# Autodesk Inventor assembly: 000-dribl-v2
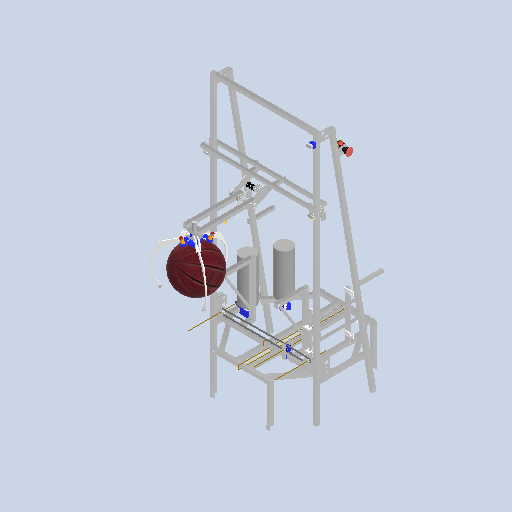
[picture p0: Inventor's stored thumbnail of the model, 512x512]
Saved by Autodesk Inventor 2025.2 (Build 292293000, 293)
## iProperties
Created: 2025-04-03
Part Number: 000-dribl-v2
Document SubType Name: Assembly
Designer: haruy
Author: haruy
## Documents named in this file (45)
- C:\Users\haruy\Documents\ロボコン\NHK2025\cad\nagahisa\dribl\000-dribl-v2.iam
- C:\Users\haruy\Documents\ロボコン\NHK2025\cad\nagahisa\dribl\dribl-v3-Sketch-Base.ipt
- C:\Users\haruy\Documents\ロボコン\NHK2025\cad\nagahisa\dribl\dribl-v1-Plate-5.ipt
- C:\Users\haruy\Documents\ロボコン\NHK2025\cad\nagahisa\dribl\dribl-v1-Plate-3.ipt
- C:\Users\haruy\Documents\ロボコン\NHK2025\cad\nagahisa\dribl\dribl-v1-Plate-4.ipt
- C:\Users\haruy\Documents\ロボコン\NHK2025\cad\nagahisa\dribl\dribl-v3-Plate-1.ipt
- C:\Users\haruy\Documents\ロボコン\NHK2025\cad\nagahisa\dribl\dribl-v3-Plate-2.ipt
- C:\Users\haruy\Documents\ロボコン\NHK2025\cad\nagahisa\dribl\dribl-v3-ASP-arm.ipt
- C:\Users\haruy\Documents\ロボコン\NHK2025\cad\nagahisa\dribl\dribl-v3-Plate-3.ipt
- C:\Users\haruy\Documents\ロボコン\NHK2025\cad\nagahisa\dribl\dribl-v1-Shaft-spesa-57.ipt
- C:\Users\haruy\Documents\ロボコン\NHK2025\cad\nagahisa\dribl\dribl-v3-Plate-4.ipt
- C:\Users\haruy\Documents\ロボコン\NHK2025\cad\nagahisa\dribl\dribl-v1-Plate-8.ipt
- C:\Users\haruy\Documents\ロボコン\NHK2025\cad\000_parts\モーター\robomaster\M2006 P36\RoboMaster M2006 P36\RoboMaster M2006 P36.ipt
- C:\Users\haruy\Documents\ロボコン\NHK2025\cad\nagahisa\dribl\dribl-v3-Plate-6.ipt
- C:\Users\haruy\Documents\ロボコン\NHK2025\cad\nagahisa\dribl\dribl-v3-Plate-7.ipt
- C:\Users\haruy\Documents\ロボコン\NHK2025\cad\nagahisa\dribl\dribl-v3-Plate-8.ipt
- C:\Users\haruy\Documents\ロボコン\NHK2025\cad\nagahisa\dribl\dribl-v3-Plate-9.ipt
- C:\Users\haruy\Documents\ロボコン\NHK2025\cad\nagahisa\dribl\dribl-v3-Plate-10.ipt
- C:\Users\haruy\Documents\ロボコン\NHK2025\cad\nagahisa\dribl\dribl-v3-Plate-11.ipt
- C:\Users\haruy\Documents\ロボコン\NHK2025\cad\nagahisa\dribl\dribl-v3-Plate-12.ipt
- C:\Users\haruy\Documents\ロボコン\NHK2025\cad\nagahisa\dribl\dribl-v3-ASP-1.ipt
- C:\Users\haruy\Documents\ロボコン\NHK2025\cad\nagahisa\dribl\dribl-v1-Plate-14.ipt
- C:\Users\haruy\Documents\ロボコン\NHK2025\cad\nagahisa\dribl\dribl-v1-3DP-P-F.ipt
- C:\Users\haruy\Documents\ロボコン\NHK2025\cad\nagahisa\dribl\roller-Base-v1-petbottle.ipt
- C:\Users\haruy\Documents\ロボコン\NHK2025\cad\nagahisa\dribl\dribl-v3-Plate-13.ipt
- C:\Users\haruy\Documents\ロボコン\NHK2025\cad\nagahisa\dribl\dribl-v3-Plate-14.ipt
- C:\Users\haruy\Documents\ロボコン\NHK2025\cad\nagahisa\base_weel\base_weel-v2-Plate-8.ipt
- C:\Users\haruy\Documents\ロボコン\NHK2025\cad\nagahisa\dribl\dribl-v3-ASP-2.ipt
- C:\Users\haruy\Documents\ロボコン\NHK2025\cad\nagahisa\base_weel\base_weel-v2-POM-pc-F-1.ipt
- C:\Users\haruy\Documents\ロボコン\NHK2025\cad\nagahisa\base_weel\base_weel-v2-POM-pc-F-2.ipt
- C:\Users\haruy\Documents\ロボコン\NHK2025\cad\nagahisa\dribl\dribl-v3-Plate-15.ipt
- C:\Users\haruy\Documents\ロボコン\NHK2025\cad\nagahisa\dribl\dribl-v1-Plate-13.ipt
- C:\Users\haruy\Documents\ロボコン\NHK2025\cad\000_parts\回路関連\EMO\emo_sa.ipt
- C:\Users\haruy\Documents\ロボコン\NHK2025\cad\nagahisa\dribl\dribl-v3-3DP-1.ipt
- C:\Users\haruy\Documents\ロボコン\NHK2025\cad\nagahisa\dribl\dribl-v3-Plate-16.ipt
- C:\Users\haruy\Documents\ロボコン\NHK2025\cad\nagahisa\dribl\000-dribl-v2\デザイン アクセラレータ\歯付きベルト伝達1.iam
- C:\Users\haruy\Documents\ロボコン\NHK2025\cad\000_parts\ベアリング\10\bear_10_15_sn.ipt
- C:\Users\haruy\Documents\ロボコン\NHK2025\cad\nagahisa\belt_liner\SCBRJ10-13.iam
- C:\Users\haruy\Documents\ロボコン\NHK2025\cad\nagahisa\dribl\dribl-v1-Plate-12.ipt
- C:\Users\haruy\Documents\ロボコン\NHK2025\cad\nagahisa\dribl\dribl-v1-3DP-l-F-1.ipt
- C:\Users\haruy\Documents\ロボコン\NHK2025\cad\000_parts\センサー\VX-012-1A3\VX-012-1A3\VX-012-1A3.iam
- C:\Users\haruy\Documents\ロボコン\NHK2025\cad\nagahisa\dribl\R2-Rzvector\TH22_bearing_12_18_19.5_sn.ipt
- C:\Users\haruy\Documents\ロボコン\NHK2025\cad\nagahisa\dribl\SCSNAJ12-16b.ipt
- C:\Users\haruy\Documents\ロボコン\NHK2025\cad\nagahisa\dribl\dribl-v1-Shaft-2.ipt
- C:\Users\haruy\Documents\ロボコン\NHK2025\cad\nagahisa\hand\grab\000-hand-grab-v4.iam
## Components (87 placed, 44 different names)
1. dribl-v3-Sketch-Base:1 — 挿入:10, 挿入:11, 挿入:12, 挿入:13, 挿入:14, 挿入:15, 挿入:16, 挿入:17, 挿入:18, 挿入:19, 挿入:20, 挿入:21, 挿入:22, 挿入:23, 挿入:24, 挿入:25, 挿入:26, 挿入:27, 挿入:28, 挿入:29, 挿入:30, 挿入:31, 挿入:32, 挿入:33, 正接:1, 正接:2, 正接:3, 正接:4, 挿入:44, 挿入:45, 挿入:46, 挿入:47, 挿入:48, 挿入:49, 挿入:50, 挿入:51, 挿入:52, 挿入:53, 挿入:56, 挿入:57, 挿入:58, 挿入:59, 挿入:60, 挿入:61, 挿入:62, 挿入:63, 挿入:64, 挿入:65, 挿入:70, 挿入:71, 挿入:72, 挿入:73, 挿入:74, 挿入:75, 挿入:76, 挿入:77, 挿入:78, 挿入:79, 挿入:80, 挿入:81, 挿入:82, 挿入:83, 挿入:84, 挿入:85, 挿入:86, 挿入:87, 挿入:88, 挿入:89, 挿入:90, 挿入:91, 挿入:92, 挿入:93, 挿入:94, 挿入:95, 挿入:96, 挿入:97, メイト:3, メイト:4, メイト:5, メイト:6, 挿入:102, 挿入:103, 挿入:104, 挿入:105, 挿入:106, 挿入:107, 挿入:108, 挿入:109, 挿入:128, 挿入:129, 挿入:130, 挿入:131, 挿入:132, 挿入:133, 挿入:134, 挿入:135, 挿入:137, 挿入:138, 挿入:139, 挿入:140, フラッシュ:1, 挿入:149, 挿入:150, 挿入:151, 挿入:152
2. dribl-v1-Plate-5:1 — 挿入:12, 挿入:13
3. dribl-v1-Plate-5:2 — 挿入:10, 挿入:11
4. dribl-v1-Plate-3:1 — 挿入:14, 挿入:15
5. dribl-v1-Plate-4:1 — 挿入:16, 挿入:17
6. dribl-v3-Plate-1:1 — 挿入:18, 挿入:19
7. dribl-v3-Plate-1:2 — 挿入:20, 挿入:21
8. dribl-v3-Plate-1:3 — 挿入:22, 挿入:23
9. dribl-v3-Plate-1:4 — 挿入:24, 挿入:25
10. dribl-v3-Plate-2:1 — 挿入:26, 挿入:27
11. dribl-v3-Plate-2:2 — 挿入:28, 挿入:29
12. dribl-v3-Plate-2:3 — 挿入:32, 挿入:33
13. dribl-v3-Plate-2:4 — 挿入:30, 挿入:31
14. dribl-v3-ASP-arm:1 — 正接:1, 正接:2, 正接:3, 正接:4, 挿入:34, 挿入:35, 挿入:37, 挿入:38, メイト:7, 角度:1
15. dribl-v3-Plate-3:1 — 挿入:34, 挿入:35, 挿入:36, 挿入:39, 挿入:40, 挿入:158
16. dribl-v1-Shaft-spesa-57:1 — 挿入:36, 挿入:41
17. dribl-v3-Plate-4:1 — 挿入:37, 挿入:38, 挿入:157
18. dribl-v1-Shaft-spesa-57:2 — 挿入:40
19. dribl-v1-Shaft-spesa-57:3 — 挿入:39, 挿入:42
20. dribl-v1-Plate-8:1 — 挿入:41, 挿入:42, 挿入:43
21. RoboMaster M2006 P36:1 — 挿入:43
22. dribl-v3-Plate-6:1 — 挿入:44, 挿入:45
23. dribl-v3-Plate-6:2 — 挿入:50, 挿入:51
24. dribl-v3-Plate-6:3 — 挿入:48, 挿入:49
25. dribl-v3-Plate-6:4 — 挿入:46, 挿入:47
26. dribl-v3-Plate-7:1 — 挿入:52, 挿入:53
27. dribl-v3-Plate-7:4 — 挿入:56, 挿入:57
28. dribl-v3-Plate-8:1 — 挿入:58, 挿入:59
29. dribl-v3-Plate-8:2 — 挿入:60, 挿入:61
30. dribl-v3-Plate-9:1 — 挿入:62, 挿入:63
31. dribl-v3-Plate-9:3 — 挿入:64, 挿入:65
32. dribl-v3-Plate-10:1 — 挿入:72, 挿入:73
33. dribl-v3-Plate-10:2 — 挿入:74, 挿入:75
34. dribl-v3-Plate-10:3 — 挿入:70, 挿入:71
35. dribl-v3-Plate-10:4 — 挿入:76, 挿入:77
36. dribl-v3-Plate-11:1 — 挿入:78, 挿入:79
37. dribl-v3-Plate-11:2 — 挿入:82, 挿入:83
38. dribl-v3-Plate-11:3 — 挿入:80, 挿入:81
39. dribl-v3-Plate-11:4 — 挿入:84, 挿入:85
40. dribl-v3-Plate-11:5 — 挿入:88, 挿入:89
41. dribl-v3-Plate-11:6 — 挿入:86, 挿入:87
42. dribl-v3-Plate-12:1 — 挿入:90, 挿入:91
43. dribl-v3-Plate-12:2 — 挿入:92, 挿入:93
44. dribl-v3-ASP-1:1 — 挿入:98, 挿入:99
45. dribl-v1-Plate-14:1 — 挿入:96, 挿入:97
46. dribl-v1-Plate-14:2 — 挿入:94, 挿入:95, 挿入:98, 挿入:99
47. dribl-v1-3DP-P-F:1 — 挿入:100, メイト:5, メイト:6
48. roller-Base-v1-petbottle:1 — 挿入:100
49. dribl-v1-3DP-P-F:2 — メイト:3, メイト:4, 挿入:101
50. roller-Base-v1-petbottle:2 — 挿入:101
51. dribl-v3-Plate-13:1 — 挿入:102, 挿入:103
52. dribl-v3-Plate-14:1 — 挿入:104, 挿入:105
53. base_weel-v2-Plate-8:1 — 挿入:106, 挿入:107, 挿入:110, 挿入:111
54. base_weel-v2-Plate-8:2 — 挿入:108, 挿入:109
55. dribl-v3-ASP-2:1 — 挿入:110, 挿入:111, 挿入:112, 挿入:113, 挿入:114, 挿入:115, 挿入:116, 挿入:117, 挿入:118, 挿入:119, 挿入:120, 挿入:121, 挿入:122, 挿入:123, 挿入:124, 挿入:125, 挿入:126, 挿入:127
56. base_weel-v2-POM-pc-F-1:1 — 挿入:112, 挿入:113
57. base_weel-v2-POM-pc-F-1:2 — 挿入:114, 挿入:115
58. base_weel-v2-POM-pc-F-2:1 — 挿入:118, 挿入:119
59. base_weel-v2-POM-pc-F-2:2 — 挿入:116, 挿入:117
60. base_weel-v2-POM-pc-F-2:3 — 挿入:122, 挿入:123
61. base_weel-v2-POM-pc-F-2:4 — 挿入:120, 挿入:121
62. base_weel-v2-POM-pc-F-1:3 — 挿入:126, 挿入:127
63. base_weel-v2-POM-pc-F-1:4 — 挿入:124, 挿入:125
64. dribl-v3-Plate-15:1 — 挿入:128, 挿入:129
65. dribl-v3-Plate-15:2 — 挿入:130, 挿入:131
66. dribl-v3-Plate-11:7 — 挿入:132, 挿入:133
67. dribl-v1-Plate-13:1 — 挿入:134, 挿入:135, 挿入:136
68. emo_sa:1 — 挿入:136
69. dribl-v3-3DP-1:1 — 挿入:139, 挿入:140, 挿入:143, 挿入:144
70. dribl-v3-3DP-1:2 — 挿入:137, 挿入:138, 挿入:141, 挿入:142
71. dribl-v3-Plate-16:1 — 挿入:143, 挿入:144
72. dribl-v3-Plate-16:2 — 挿入:141, 挿入:142
73. 歯付きベルト伝達:1 [sub-assembly] — 挿入:145, 挿入:146
74. bear_10_15_sn:1 — 挿入:145, 挿入:147
75. bear_10_15_sn:2 — 挿入:146, 挿入:148
76. SCBRJ10-13:1 [sub-assembly] — 挿入:147
77. SCBRJ10-13:2 [sub-assembly] — 挿入:148
78. dribl-v1-Plate-12:1 — 挿入:149, 挿入:150, 挿入:155, 挿入:156
79. dribl-v1-3DP-l-F-1:1 — 挿入:151, 挿入:152, 挿入:153, 挿入:154
80. VX-012-1A3:1 [sub-assembly] — 挿入:153, 挿入:154
81. VX-012-1A3:2 [sub-assembly] — 挿入:155, 挿入:156, メイト:7
82. TH22_bearing_12_18_19.5_sn:1 — 挿入:157, 挿入:160
83. TH22_bearing_12_18_19.5_sn:2 — 挿入:158, 挿入:159, 挿入:162
84. SCSNAJ12-16b:1 — 挿入:159, 挿入:161
85. SCSNAJ12-16b:2 — 挿入:160
86. dribl-v1-Shaft-2:1 — 挿入:161
87. 000-hand-grab-v4:1 [sub-assembly] — 挿入:162, 角度:1
## Relationships (158: Insert 147, Mate 5, Tangent 4, Flush 1, Angle 1)
- 挿入:10 [Insert]: dribl-v3-Sketch-Base:1 ↔ dribl-v1-Plate-5:2
- 挿入:11 [Insert]: dribl-v3-Sketch-Base:1 ↔ dribl-v1-Plate-5:2
- 挿入:12 [Insert]: dribl-v3-Sketch-Base:1 ↔ dribl-v1-Plate-5:1
- 挿入:13 [Insert]: dribl-v3-Sketch-Base:1 ↔ dribl-v1-Plate-5:1
- 挿入:14 [Insert]: dribl-v3-Sketch-Base:1 ↔ dribl-v1-Plate-3:1
- 挿入:15 [Insert]: dribl-v3-Sketch-Base:1 ↔ dribl-v1-Plate-3:1
- 挿入:16 [Insert]: dribl-v3-Sketch-Base:1 ↔ dribl-v1-Plate-4:1
- 挿入:17 [Insert]: dribl-v3-Sketch-Base:1 ↔ dribl-v1-Plate-4:1
- 挿入:18 [Insert]: dribl-v3-Sketch-Base:1 ↔ dribl-v3-Plate-1:1
- 挿入:19 [Insert]: dribl-v3-Sketch-Base:1 ↔ dribl-v3-Plate-1:1
- 挿入:20 [Insert]: dribl-v3-Sketch-Base:1 ↔ dribl-v3-Plate-1:2
- 挿入:21 [Insert]: dribl-v3-Sketch-Base:1 ↔ dribl-v3-Plate-1:2
- 挿入:22 [Insert]: dribl-v3-Sketch-Base:1 ↔ dribl-v3-Plate-1:3
- 挿入:23 [Insert]: dribl-v3-Sketch-Base:1 ↔ dribl-v3-Plate-1:3
- 挿入:24 [Insert]: dribl-v3-Sketch-Base:1 ↔ dribl-v3-Plate-1:4
- 挿入:25 [Insert]: dribl-v3-Sketch-Base:1 ↔ dribl-v3-Plate-1:4
- 挿入:26 [Insert]: dribl-v3-Sketch-Base:1 ↔ dribl-v3-Plate-2:1
- 挿入:27 [Insert]: dribl-v3-Sketch-Base:1 ↔ dribl-v3-Plate-2:1
- 挿入:28 [Insert]: dribl-v3-Sketch-Base:1 ↔ dribl-v3-Plate-2:2
- 挿入:29 [Insert]: dribl-v3-Sketch-Base:1 ↔ dribl-v3-Plate-2:2
- 挿入:30 [Insert]: dribl-v3-Sketch-Base:1 ↔ dribl-v3-Plate-2:4
- 挿入:31 [Insert]: dribl-v3-Sketch-Base:1 ↔ dribl-v3-Plate-2:4
- 挿入:32 [Insert]: dribl-v3-Sketch-Base:1 ↔ dribl-v3-Plate-2:3
- 挿入:33 [Insert]: dribl-v3-Sketch-Base:1 ↔ dribl-v3-Plate-2:3
- 正接:1 [Tangent]: dribl-v3-Sketch-Base:1 ↔ dribl-v3-ASP-arm:1
- 正接:2 [Tangent]: dribl-v3-Sketch-Base:1 ↔ dribl-v3-ASP-arm:1
- 正接:3 [Tangent]: dribl-v3-Sketch-Base:1 ↔ dribl-v3-ASP-arm:1
- 正接:4 [Tangent]: dribl-v3-Sketch-Base:1 ↔ dribl-v3-ASP-arm:1
- 挿入:34 [Insert]: dribl-v3-ASP-arm:1 ↔ dribl-v3-Plate-3:1
- 挿入:35 [Insert]: dribl-v3-ASP-arm:1 ↔ dribl-v3-Plate-3:1
- 挿入:36 [Insert]: dribl-v3-Plate-3:1 ↔ dribl-v1-Shaft-spesa-57:1
- 挿入:37 [Insert]: dribl-v3-ASP-arm:1 ↔ dribl-v3-Plate-4:1
- 挿入:38 [Insert]: dribl-v3-ASP-arm:1 ↔ dribl-v3-Plate-4:1
- 挿入:39 [Insert]: dribl-v3-Plate-3:1 ↔ dribl-v1-Shaft-spesa-57:3
- 挿入:40 [Insert]: dribl-v3-Plate-3:1 ↔ dribl-v1-Shaft-spesa-57:2
- 挿入:41 [Insert]: dribl-v1-Shaft-spesa-57:1 ↔ dribl-v1-Plate-8:1
- 挿入:42 [Insert]: dribl-v1-Shaft-spesa-57:3 ↔ dribl-v1-Plate-8:1
- 挿入:43 [Insert]: dribl-v1-Plate-8:1 ↔ RoboMaster M2006 P36:1
- 挿入:44 [Insert]: dribl-v3-Sketch-Base:1 ↔ dribl-v3-Plate-6:1
- 挿入:45 [Insert]: dribl-v3-Sketch-Base:1 ↔ dribl-v3-Plate-6:1
- 挿入:46 [Insert]: dribl-v3-Sketch-Base:1 ↔ dribl-v3-Plate-6:4
- 挿入:47 [Insert]: dribl-v3-Sketch-Base:1 ↔ dribl-v3-Plate-6:4
- 挿入:48 [Insert]: dribl-v3-Sketch-Base:1 ↔ dribl-v3-Plate-6:3
- 挿入:49 [Insert]: dribl-v3-Sketch-Base:1 ↔ dribl-v3-Plate-6:3
- 挿入:50 [Insert]: dribl-v3-Sketch-Base:1 ↔ dribl-v3-Plate-6:2
- 挿入:51 [Insert]: dribl-v3-Sketch-Base:1 ↔ dribl-v3-Plate-6:2
- 挿入:52 [Insert]: dribl-v3-Sketch-Base:1 ↔ dribl-v3-Plate-7:1
- 挿入:53 [Insert]: dribl-v3-Sketch-Base:1 ↔ dribl-v3-Plate-7:1
- 挿入:56 [Insert]: dribl-v3-Sketch-Base:1 ↔ dribl-v3-Plate-7:4
- 挿入:57 [Insert]: dribl-v3-Sketch-Base:1 ↔ dribl-v3-Plate-7:4
- 挿入:58 [Insert]: dribl-v3-Sketch-Base:1 ↔ dribl-v3-Plate-8:1
- 挿入:59 [Insert]: dribl-v3-Sketch-Base:1 ↔ dribl-v3-Plate-8:1
- 挿入:60 [Insert]: dribl-v3-Sketch-Base:1 ↔ dribl-v3-Plate-8:2
- 挿入:61 [Insert]: dribl-v3-Sketch-Base:1 ↔ dribl-v3-Plate-8:2
- 挿入:62 [Insert]: dribl-v3-Sketch-Base:1 ↔ dribl-v3-Plate-9:1
- 挿入:63 [Insert]: dribl-v3-Sketch-Base:1 ↔ dribl-v3-Plate-9:1
- 挿入:64 [Insert]: dribl-v3-Sketch-Base:1 ↔ dribl-v3-Plate-9:3
- 挿入:65 [Insert]: dribl-v3-Sketch-Base:1 ↔ dribl-v3-Plate-9:3
- 挿入:70 [Insert]: dribl-v3-Sketch-Base:1 ↔ dribl-v3-Plate-10:3
- 挿入:71 [Insert]: dribl-v3-Sketch-Base:1 ↔ dribl-v3-Plate-10:3
- 挿入:72 [Insert]: dribl-v3-Sketch-Base:1 ↔ dribl-v3-Plate-10:1
- 挿入:73 [Insert]: dribl-v3-Sketch-Base:1 ↔ dribl-v3-Plate-10:1
- 挿入:74 [Insert]: dribl-v3-Sketch-Base:1 ↔ dribl-v3-Plate-10:2
- 挿入:75 [Insert]: dribl-v3-Sketch-Base:1 ↔ dribl-v3-Plate-10:2
- 挿入:76 [Insert]: dribl-v3-Sketch-Base:1 ↔ dribl-v3-Plate-10:4
- 挿入:77 [Insert]: dribl-v3-Sketch-Base:1 ↔ dribl-v3-Plate-10:4
- 挿入:78 [Insert]: dribl-v3-Sketch-Base:1 ↔ dribl-v3-Plate-11:1
- 挿入:79 [Insert]: dribl-v3-Sketch-Base:1 ↔ dribl-v3-Plate-11:1
- 挿入:80 [Insert]: dribl-v3-Sketch-Base:1 ↔ dribl-v3-Plate-11:3
- 挿入:81 [Insert]: dribl-v3-Sketch-Base:1 ↔ dribl-v3-Plate-11:3
- 挿入:82 [Insert]: dribl-v3-Sketch-Base:1 ↔ dribl-v3-Plate-11:2
- 挿入:83 [Insert]: dribl-v3-Sketch-Base:1 ↔ dribl-v3-Plate-11:2
- 挿入:84 [Insert]: dribl-v3-Sketch-Base:1 ↔ dribl-v3-Plate-11:4
- 挿入:85 [Insert]: dribl-v3-Sketch-Base:1 ↔ dribl-v3-Plate-11:4
- 挿入:86 [Insert]: dribl-v3-Sketch-Base:1 ↔ dribl-v3-Plate-11:6
- 挿入:87 [Insert]: dribl-v3-Sketch-Base:1 ↔ dribl-v3-Plate-11:6
- 挿入:88 [Insert]: dribl-v3-Sketch-Base:1 ↔ dribl-v3-Plate-11:5
- 挿入:89 [Insert]: dribl-v3-Sketch-Base:1 ↔ dribl-v3-Plate-11:5
- 挿入:90 [Insert]: dribl-v3-Sketch-Base:1 ↔ dribl-v3-Plate-12:1
- 挿入:91 [Insert]: dribl-v3-Sketch-Base:1 ↔ dribl-v3-Plate-12:1
- 挿入:92 [Insert]: dribl-v3-Sketch-Base:1 ↔ dribl-v3-Plate-12:2
- 挿入:93 [Insert]: dribl-v3-Sketch-Base:1 ↔ dribl-v3-Plate-12:2
- 挿入:94 [Insert]: dribl-v3-Sketch-Base:1 ↔ dribl-v1-Plate-14:2
- 挿入:95 [Insert]: dribl-v3-Sketch-Base:1 ↔ dribl-v1-Plate-14:2
- 挿入:96 [Insert]: dribl-v3-Sketch-Base:1 ↔ dribl-v1-Plate-14:1
- 挿入:97 [Insert]: dribl-v3-Sketch-Base:1 ↔ dribl-v1-Plate-14:1
- 挿入:98 [Insert]: dribl-v3-ASP-1:1 ↔ dribl-v1-Plate-14:2
- 挿入:99 [Insert]: dribl-v3-ASP-1:1 ↔ dribl-v1-Plate-14:2
- 挿入:100 [Insert]: dribl-v1-3DP-P-F:1 ↔ roller-Base-v1-petbottle:1
- メイト:3 [Mate]: dribl-v3-Sketch-Base:1 ↔ dribl-v1-3DP-P-F:2
- メイト:4 [Mate]: dribl-v3-Sketch-Base:1 ↔ dribl-v1-3DP-P-F:2
- 挿入:101 [Insert]: dribl-v1-3DP-P-F:2 ↔ roller-Base-v1-petbottle:2
- メイト:5 [Mate]: dribl-v3-Sketch-Base:1 ↔ dribl-v1-3DP-P-F:1
- メイト:6 [Mate]: dribl-v3-Sketch-Base:1 ↔ dribl-v1-3DP-P-F:1
- 挿入:102 [Insert]: dribl-v3-Sketch-Base:1 ↔ dribl-v3-Plate-13:1
- 挿入:103 [Insert]: dribl-v3-Sketch-Base:1 ↔ dribl-v3-Plate-13:1
- 挿入:104 [Insert]: dribl-v3-Sketch-Base:1 ↔ dribl-v3-Plate-14:1
- 挿入:105 [Insert]: dribl-v3-Sketch-Base:1 ↔ dribl-v3-Plate-14:1
- 挿入:106 [Insert]: dribl-v3-Sketch-Base:1 ↔ base_weel-v2-Plate-8:1
- 挿入:107 [Insert]: dribl-v3-Sketch-Base:1 ↔ base_weel-v2-Plate-8:1
- 挿入:108 [Insert]: dribl-v3-Sketch-Base:1 ↔ base_weel-v2-Plate-8:2
- 挿入:109 [Insert]: dribl-v3-Sketch-Base:1 ↔ base_weel-v2-Plate-8:2
- 挿入:110 [Insert]: base_weel-v2-Plate-8:1 ↔ dribl-v3-ASP-2:1
- 挿入:111 [Insert]: base_weel-v2-Plate-8:1 ↔ dribl-v3-ASP-2:1
- 挿入:112 [Insert]: dribl-v3-ASP-2:1 ↔ base_weel-v2-POM-pc-F-1:1
- 挿入:113 [Insert]: dribl-v3-ASP-2:1 ↔ base_weel-v2-POM-pc-F-1:1
- 挿入:114 [Insert]: dribl-v3-ASP-2:1 ↔ base_weel-v2-POM-pc-F-1:2
- 挿入:115 [Insert]: dribl-v3-ASP-2:1 ↔ base_weel-v2-POM-pc-F-1:2
- 挿入:116 [Insert]: dribl-v3-ASP-2:1 ↔ base_weel-v2-POM-pc-F-2:2
- 挿入:117 [Insert]: dribl-v3-ASP-2:1 ↔ base_weel-v2-POM-pc-F-2:2
- 挿入:118 [Insert]: dribl-v3-ASP-2:1 ↔ base_weel-v2-POM-pc-F-2:1
- 挿入:119 [Insert]: dribl-v3-ASP-2:1 ↔ base_weel-v2-POM-pc-F-2:1
- 挿入:120 [Insert]: dribl-v3-ASP-2:1 ↔ base_weel-v2-POM-pc-F-2:4
- 挿入:121 [Insert]: dribl-v3-ASP-2:1 ↔ base_weel-v2-POM-pc-F-2:4
- 挿入:122 [Insert]: dribl-v3-ASP-2:1 ↔ base_weel-v2-POM-pc-F-2:3
- 挿入:123 [Insert]: dribl-v3-ASP-2:1 ↔ base_weel-v2-POM-pc-F-2:3
- 挿入:124 [Insert]: dribl-v3-ASP-2:1 ↔ base_weel-v2-POM-pc-F-1:4
- 挿入:125 [Insert]: dribl-v3-ASP-2:1 ↔ base_weel-v2-POM-pc-F-1:4
- 挿入:126 [Insert]: dribl-v3-ASP-2:1 ↔ base_weel-v2-POM-pc-F-1:3
- 挿入:127 [Insert]: dribl-v3-ASP-2:1 ↔ base_weel-v2-POM-pc-F-1:3
- 挿入:128 [Insert]: dribl-v3-Sketch-Base:1 ↔ dribl-v3-Plate-15:1
- 挿入:129 [Insert]: dribl-v3-Sketch-Base:1 ↔ dribl-v3-Plate-15:1
- 挿入:130 [Insert]: dribl-v3-Sketch-Base:1 ↔ dribl-v3-Plate-15:2
- 挿入:131 [Insert]: dribl-v3-Sketch-Base:1 ↔ dribl-v3-Plate-15:2
- 挿入:132 [Insert]: dribl-v3-Sketch-Base:1 ↔ dribl-v3-Plate-11:7
- 挿入:133 [Insert]: dribl-v3-Sketch-Base:1 ↔ dribl-v3-Plate-11:7
- 挿入:134 [Insert]: dribl-v3-Sketch-Base:1 ↔ dribl-v1-Plate-13:1
- 挿入:135 [Insert]: dribl-v3-Sketch-Base:1 ↔ dribl-v1-Plate-13:1
- 挿入:136 [Insert]: dribl-v1-Plate-13:1 ↔ emo_sa:1
- 挿入:137 [Insert]: dribl-v3-Sketch-Base:1 ↔ dribl-v3-3DP-1:2
- 挿入:138 [Insert]: dribl-v3-Sketch-Base:1 ↔ dribl-v3-3DP-1:2
- 挿入:139 [Insert]: dribl-v3-Sketch-Base:1 ↔ dribl-v3-3DP-1:1
- 挿入:140 [Insert]: dribl-v3-Sketch-Base:1 ↔ dribl-v3-3DP-1:1
- 挿入:141 [Insert]: dribl-v3-3DP-1:2 ↔ dribl-v3-Plate-16:2
- 挿入:142 [Insert]: dribl-v3-3DP-1:2 ↔ dribl-v3-Plate-16:2
- 挿入:143 [Insert]: dribl-v3-3DP-1:1 ↔ dribl-v3-Plate-16:1
- 挿入:144 [Insert]: dribl-v3-3DP-1:1 ↔ dribl-v3-Plate-16:1
- フラッシュ:1 [Flush] (-10 mm): dribl-v3-Sketch-Base:1
- 挿入:145 [Insert]: 歯付きベルト伝達:1 ↔ bear_10_15_sn:1
- 挿入:146 [Insert]: 歯付きベルト伝達:1 ↔ bear_10_15_sn:2
- 挿入:147 [Insert]: bear_10_15_sn:1 ↔ SCBRJ10-13:1
- 挿入:148 [Insert]: bear_10_15_sn:2 ↔ SCBRJ10-13:2
- 挿入:149 [Insert]: dribl-v3-Sketch-Base:1 ↔ dribl-v1-Plate-12:1
- 挿入:150 [Insert]: dribl-v3-Sketch-Base:1 ↔ dribl-v1-Plate-12:1
- 挿入:151 [Insert]: dribl-v3-Sketch-Base:1 ↔ dribl-v1-3DP-l-F-1:1
- 挿入:152 [Insert]: dribl-v3-Sketch-Base:1 ↔ dribl-v1-3DP-l-F-1:1
- 挿入:153 [Insert]: dribl-v1-3DP-l-F-1:1 ↔ VX-012-1A3:1
- 挿入:154 [Insert]: dribl-v1-3DP-l-F-1:1 ↔ VX-012-1A3:1
- 挿入:155 [Insert]: dribl-v1-Plate-12:1 ↔ VX-012-1A3:2
- 挿入:156 [Insert]: dribl-v1-Plate-12:1 ↔ VX-012-1A3:2
- 挿入:157 [Insert]: dribl-v3-Plate-4:1 ↔ TH22_bearing_12_18_19.5_sn:1
- 挿入:158 [Insert]: dribl-v3-Plate-3:1 ↔ TH22_bearing_12_18_19.5_sn:2
- 挿入:159 [Insert]: TH22_bearing_12_18_19.5_sn:2 ↔ SCSNAJ12-16b:1
- 挿入:160 [Insert]: TH22_bearing_12_18_19.5_sn:1 ↔ SCSNAJ12-16b:2
- 挿入:161 [Insert]: SCSNAJ12-16b:1 ↔ dribl-v1-Shaft-2:1
- 挿入:162 [Insert] (11 mm): TH22_bearing_12_18_19.5_sn:2 ↔ 000-hand-grab-v4:1
- メイト:7 [Mate]: dribl-v3-ASP-arm:1 ↔ VX-012-1A3:2
- 角度:1 [Angle] (180 deg): dribl-v3-ASP-arm:1 ↔ 000-hand-grab-v4:1
